# Autodesk Inventor assembly: model-c_full
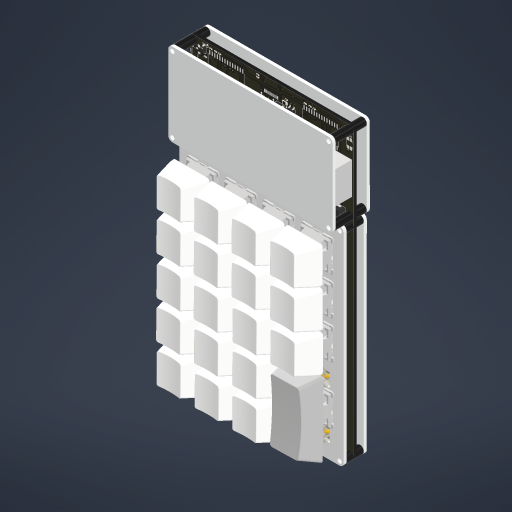
[picture p0: Inventor's stored thumbnail of the model, 512x512]
Saved by Autodesk Inventor 2024.2 (Build 282272000, 272)
## iProperties
Created: 2025-05-21
Part Number: model-c_full
Document SubType Name: Assembly
Designer: Moe
Author: Moe
## Documents named in this file (15)
- D:\Code\git\Model-C\case\model-c_full.iam
- D:\Code\git\Model-C\case\model-c.ipt
- D:\Code\git\Model-C\case\switchplate_spacer.ipt
- D:\Code\git\Model-C\case\screen_spacer.ipt
- D:\Code\git\Model-C\case\black_screen.ipt
- D:\Code\git\Model-C\case\battery_cover.ipt
- D:\Code\git\Model-C\case\switchplate.ipt
- D:\Code\git\Model-C\case\backplate.ipt
- D:\Code\git\Model-C\case\battery_spacer.ipt
- D:\Code\git\Model-C\case\14seg_surrogate.ipt
- D:\Code\git\Model-C\case\battery_surrogate.ipt
- D:\Code\git\Model-C\case\references\2U Stabilizer.ipt
- D:\Code\git\Model-C\case\references\asm_mx_asm_PCB.ipt
- D:\Code\git\Model-C\case\references\keycap.ipt
- D:\Code\git\Model-C\case\references\POS_2u_Cherry_row1.ipt
## Components (63 placed, 14 different names)
1. battery_surrogate:1 — Mate:61
2. 2U Stabilizer:1 — Mate:62
3. keycap:1
4. POS_2u_Cherry_row1:1
5. keycap:2
6. keycap:3
7. keycap:4
8. keycap:5
9. keycap:6
10. keycap:7
11. keycap:8
12. keycap:9
13. keycap:10
14. keycap:11
15. keycap:12
16. keycap:13
17. keycap:14
18. keycap:15
19. keycap:16
20. keycap:17
21. keycap:18
22. backplate:1 — Mate:47, Mate:48
23. switchplate:1 — Mate:45, Mate:46
24. battery_cover:1 — Mate:57, Mate:58
25. model-c:1 — Mate:3, Mate:4, Mate:6, Mate:8, Mate:10, Mate:12, Mate:14, Mate:16, Mate:17, Mate:18, Mate:19, Mate:20, Mate:21, Mate:22, Mate:23, Mate:24, Mate:25, Mate:26, Mate:27, Mate:28, Mate:34, Mate:36, Mate:38, Mate:40, Mate:49, Mate:50, Mate:51, Mate:52, Mate:53, Mate:54, Mate:55, Mate:56, Mate:59, Mate:60, Mate:61, Mate:62, Mate:63, Mate:64, Mate:65, Mate:66, Mate:67, Mate:68, Mate:69, Mate:70, Mate:71, Mate:72, Mate:73, Mate:74, Mate:75, Mate:76, Mate:77, Mate:78, Mate:79, Mate:80, Mate:81
26. black_screen:1 — Mate:41, Mate:42
27. asm_mx_asm_PCB:1 — Mate:78
28. asm_mx_asm_PCB:2 — Mate:76
29. asm_mx_asm_PCB:3 — Mate:75
30. asm_mx_asm_PCB:4 — Mate:81
31. asm_mx_asm_PCB:5 — Mate:80
32. asm_mx_asm_PCB:6 — Mate:79
33. asm_mx_asm_PCB:7 — Mate:73
34. asm_mx_asm_PCB:8 — Mate:72
35. asm_mx_asm_PCB:9 — Mate:71
36. asm_mx_asm_PCB:10 — Mate:70
37. asm_mx_asm_PCB:11 — Mate:69
38. asm_mx_asm_PCB:12 — Mate:68
39. asm_mx_asm_PCB:13 — Mate:67
40. asm_mx_asm_PCB:14 — Mate:66
41. asm_mx_asm_PCB:15 — Mate:65
42. asm_mx_asm_PCB:16 — Mate:63
43. asm_mx_asm_PCB:17 — Mate:64
44. asm_mx_asm_PCB:18 — Mate:74
45. asm_mx_asm_PCB:19 — Mate:77
46. battery_spacer:1 — Mate:49, Mate:50, Mate:57
47. battery_spacer:2 — Mate:51, Mate:56
48. battery_spacer:3 — Mate:52, Mate:55
49. battery_spacer:4 — Mate:53, Mate:54, Mate:58
50. switchplate_spacer:11 — Mate:17, Mate:19, Mate:48
51. switchplate_spacer:12 — Mate:18, Mate:20
52. switchplate_spacer:14 — Mate:22, Mate:23
53. switchplate_spacer:15 — Mate:21, Mate:24, Mate:46
54. switchplate_spacer:9 — Mate:10, Mate:16
55. switchplate_spacer:6 — Mate:3, Mate:4, Mate:47
56. switchplate_spacer:4 — Mate:6, Mate:8
57. switchplate_spacer:10 — Mate:12, Mate:14, Mate:45
58. screen_spacer:1 — Mate:28, Mate:36, Mate:41
59. screen_spacer:3 — Mate:27, Mate:34
60. screen_spacer:4 — Mate:26, Mate:38
61. screen_spacer:8 — Mate:25, Mate:40, Mate:42
62. 14seg_surrogate:1 — Mate:59
63. 14seg_surrogate:2 — Mate:60
## Relationships (63: Mate 63)
- Mate:3: model-c:1 ↔ switchplate_spacer:6
- Mate:4: model-c:1 ↔ switchplate_spacer:6
- Mate:6: model-c:1 ↔ switchplate_spacer:4
- Mate:8: model-c:1 ↔ switchplate_spacer:4
- Mate:10: model-c:1 ↔ switchplate_spacer:9
- Mate:12: model-c:1 ↔ switchplate_spacer:10
- Mate:14: model-c:1 ↔ switchplate_spacer:10
- Mate:16: model-c:1 ↔ switchplate_spacer:9
- Mate:17: model-c:1 ↔ switchplate_spacer:11
- Mate:18: model-c:1 ↔ switchplate_spacer:12
- Mate:19: model-c:1 ↔ switchplate_spacer:11
- Mate:20: model-c:1 ↔ switchplate_spacer:12
- Mate:21: model-c:1 ↔ switchplate_spacer:15
- Mate:22: model-c:1 ↔ switchplate_spacer:14
- Mate:23: model-c:1 ↔ switchplate_spacer:14
- Mate:24: model-c:1 ↔ switchplate_spacer:15
- Mate:25: model-c:1 ↔ screen_spacer:8
- Mate:26: model-c:1 ↔ screen_spacer:4
- Mate:27: model-c:1 ↔ screen_spacer:3
- Mate:28: model-c:1 ↔ screen_spacer:1
- Mate:34: model-c:1 ↔ screen_spacer:3
- Mate:36: model-c:1 ↔ screen_spacer:1
- Mate:38: model-c:1 ↔ screen_spacer:4
- Mate:40: model-c:1 ↔ screen_spacer:8
- Mate:41: black_screen:1 ↔ screen_spacer:1
- Mate:42: black_screen:1 ↔ screen_spacer:8
- Mate:45: switchplate:1 ↔ switchplate_spacer:10
- Mate:46: switchplate:1 ↔ switchplate_spacer:15
- Mate:47: backplate:1 ↔ switchplate_spacer:6
- Mate:48: backplate:1 ↔ switchplate_spacer:11
- Mate:49: model-c:1 ↔ battery_spacer:1
- Mate:50: model-c:1 ↔ battery_spacer:1
- Mate:51: model-c:1 ↔ battery_spacer:2
- Mate:52: model-c:1 ↔ battery_spacer:3
- Mate:53: model-c:1 ↔ battery_spacer:4
- Mate:54: model-c:1 ↔ battery_spacer:4
- Mate:55: model-c:1 ↔ battery_spacer:3
- Mate:56: model-c:1 ↔ battery_spacer:2
- Mate:57: battery_cover:1 ↔ battery_spacer:1
- Mate:58: battery_cover:1 ↔ battery_spacer:4
- Mate:59: model-c:1 ↔ 14seg_surrogate:1
- Mate:60: model-c:1 ↔ 14seg_surrogate:2
- Mate:61 (0.2 mm): battery_surrogate:1 ↔ model-c:1
- Mate:62: 2U Stabilizer:1 ↔ model-c:1
- Mate:63: model-c:1 ↔ asm_mx_asm_PCB:16
- Mate:64: model-c:1 ↔ asm_mx_asm_PCB:17
- Mate:65: model-c:1 ↔ asm_mx_asm_PCB:15
- Mate:66: model-c:1 ↔ asm_mx_asm_PCB:14
- Mate:67: model-c:1 ↔ asm_mx_asm_PCB:13
- Mate:68: model-c:1 ↔ asm_mx_asm_PCB:12
- Mate:69: model-c:1 ↔ asm_mx_asm_PCB:11
- Mate:70: model-c:1 ↔ asm_mx_asm_PCB:10
- Mate:71: model-c:1 ↔ asm_mx_asm_PCB:9
- Mate:72: model-c:1 ↔ asm_mx_asm_PCB:8
- Mate:73: model-c:1 ↔ asm_mx_asm_PCB:7
- Mate:74: model-c:1 ↔ asm_mx_asm_PCB:18
- Mate:75: model-c:1 ↔ asm_mx_asm_PCB:3
- Mate:76: model-c:1 ↔ asm_mx_asm_PCB:2
- Mate:77: model-c:1 ↔ asm_mx_asm_PCB:19
- Mate:78: model-c:1 ↔ asm_mx_asm_PCB:1
- Mate:79: model-c:1 ↔ asm_mx_asm_PCB:6
- Mate:80: model-c:1 ↔ asm_mx_asm_PCB:5
- Mate:81: model-c:1 ↔ asm_mx_asm_PCB:4
